# Autodesk Inventor assembly: chair
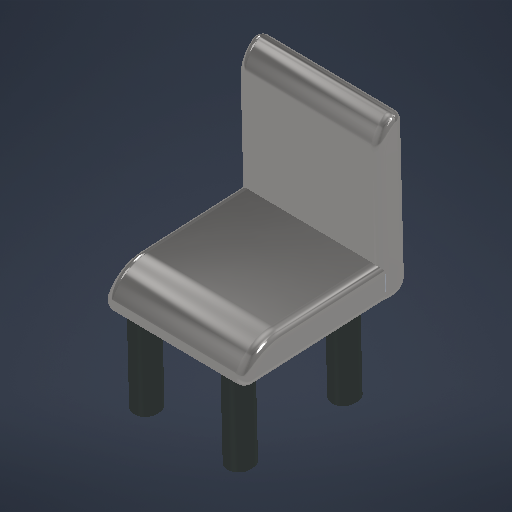
[picture p0: Inventor's stored thumbnail of the model, 512x512]
Saved by Autodesk Inventor 2027 (Build 310192000, 192)
## iProperties
Created: 2026-04-25
Part Number: chair
Document SubType Name: Assembly
Designer: sisis
Author: sisis
## Documents named in this file (4)
- C:\Users\sisis\OneDrive\Desktop\chair.iam
- C:\Users\sisis\OneDrive\Desktop\back.ipt
- C:\Users\sisis\OneDrive\Desktop\chairbase.ipt
- C:\Users\sisis\OneDrive\Desktop\leg.ipt
## Components (6 placed, 3 different names)
1. chairbase:1 — Insert:1, Insert:7, Insert:8, Insert:9, Insert:10
2. back:1 — Insert:1
3. leg:3 — Insert:7
4. leg:4 — Insert:8
5. leg:5 — Insert:9
6. leg:6 — Insert:10
## Relationships (5: Insert 5)
- Insert:1: chairbase:1 ↔ back:1
- Insert:7: chairbase:1 ↔ leg:3
- Insert:8: chairbase:1 ↔ leg:4
- Insert:9: chairbase:1 ↔ leg:5
- Insert:10: chairbase:1 ↔ leg:6
